# Autodesk Inventor assembly: Cover
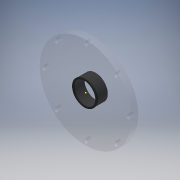
[picture p0: Inventor's stored thumbnail of the model, 180x180]
Saved by Autodesk Inventor 2017 (Build 210142000, 142)
## iProperties
Created: 2016-10-31
Part Number: Cover
Document SubType Name: Assembly
Designer: Andres
Author: Andres
## Documents named in this file (6)
- Z:\Documents\repositorios\BoreholeCamera\CAD_Probe\Enclosure\Assembly\Cover.iam
- Z:\Documents\repositorios\BoreholeCamera\CAD_Probe\Enclosure\Parts\Cover.ipt
- Z:\Documents\repositorios\BoreholeCamera\CAD_Probe\Enclosure\Parts\CoverPart1.ipt
- Z:\Documents\repositorios\BoreholeCamera\CAD_Probe\Enclosure\Parts\CoverPart2.ipt
- \\Mac\Home\Documents\repositorios\BoreholeCamera\CAD_Probe\Enclosure\Parts\CoverPart3.ipt
- \\Mac\Home\Documents\repositorios\BoreholeCamera\CAD_Probe\Enclosure\Parts\CoverPart4.ipt
## Components (5 placed, 5 different names)
1. Cover:1 — Rigid:1
2. CoverPart1:1 — Rigid:1, Rigid:2, Rigid:3, Rigid:4
3. CoverPart2:1 — Rigid:2
4. CoverPart3:1 — Rigid:3
5. CoverPart4:1 — Rigid:4
## Relationships (4: WeldJoint 4)
- Rigid:1 [WeldJoint]: Cover:1 ↔ CoverPart1:1
- Rigid:2 [WeldJoint]: CoverPart1:1 ↔ CoverPart2:1
- Rigid:3 [WeldJoint]: CoverPart1:1 ↔ CoverPart3:1
- Rigid:4 [WeldJoint]: CoverPart1:1 ↔ CoverPart4:1
